# Autodesk Inventor assembly: micromouse
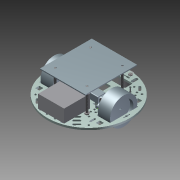
[picture p0: Inventor's stored thumbnail of the model, 180x180]
Saved by Autodesk Inventor 2015 (Build 190159000, 159)
## iProperties
Created: 2015-11-28
Part Number: micromouse
Document SubType Name: Assembly
Designer: user
Author: user
## Documents named in this file (17)
- C:\Users\user\Desktop\UNIVERSIDAD\8 SEMESTRE\FINITOS\Proyecto final\micromouse.iam
- C:\Users\user\Desktop\UNIVERSIDAD\8 SEMESTRE\FINITOS\Proyecto final\Imported Components\bracket\bracket.ipt
- C:\Users\user\Desktop\UNIVERSIDAD\8 SEMESTRE\FINITOS\Proyecto final\Imported Components\PlacaProyectoParaNX_stp\PlacaProyectoParaNX_stp.ipt
- C:\Users\user\Desktop\UNIVERSIDAD\8 SEMESTRE\FINITOS\Proyecto final\Imported Components\micromotor\micromotor.ipt
- C:\Users\user\Desktop\UNIVERSIDAD\8 SEMESTRE\FINITOS\Proyecto final\Imported Components\eje motor\eje motor.ipt
- C:\Users\user\Desktop\UNIVERSIDAD\8 SEMESTRE\FINITOS\Proyecto final\Imported Components\RuedasCaucho\RuedasCaucho.ipt
- C:\Users\user\Desktop\UNIVERSIDAD\8 SEMESTRE\FINITOS\Proyecto final\Imported Components\RuedasCentro\RuedasCentro.ipt
- C:\Users\user\Documents\Inventor\Content Center Files\R2015\es-ES\AS 1112 (4)\AS 1112 - M3(2).ipt
- C:\Users\user\Documents\Inventor\Content Center Files\R2015\es-ES\AS 1427(08)\AS 1427 - M3 x 40(6) I.ipt
- C:\Users\user\Documents\Inventor\Content Center Files\R2015\es-ES\AS 1112 (4)\AS 1112 - M1.6(2).ipt
- C:\Users\user\Documents\Inventor\Content Center Files\R2015\es-ES\BS EN ISO 7045 H\EN ISO 7045 - M1.6 x 12 - 4.8 - H(1).ipt
- C:\Users\user\Desktop\UNIVERSIDAD\8 SEMESTRE\FINITOS\Proyecto final\Imported Components\placa circuito\placa circuito.ipt
- C:\Users\user\Desktop\UNIVERSIDAD\8 SEMESTRE\FINITOS\Proyecto final\bateria.ipt
- C:\Users\user\Desktop\UNIVERSIDAD\8 SEMESTRE\FINITOS\Proyecto final\rueda loca bola.ipt
- C:\Users\user\Desktop\UNIVERSIDAD\8 SEMESTRE\FINITOS\Proyecto final\rueda loca.ipt
- C:\Users\user\Documents\Inventor\Content Center Files\R2015\es-ES\AS 1427(08)\AS 1427 - M2.5 x 25(6) I.ipt
- C:\Users\user\Documents\Inventor\Content Center Files\R2015\es-ES\AS 1112 (4)\AS 1112 - M2.5(2).ipt
## Components (39 placed, 16 different names)
1. bracket:2 — De rotación:1, Rígido:12, Insertar:11, Insertar:12
2. bracket:3 — De rotación:2, Rígido:10, Insertar:13, Insertar:14
3. PlacaProyectoParaNX_stp:1 — De rotación:1, De rotación:2, Insertar:3, Insertar:4, Insertar:5, Insertar:6, Insertar:7, Insertar:9, Insertar:10, Rígido:13, Rígido:14
4. micromotor:1 — Rígido:9, Rígido:12
5. micromotor:2 — Rígido:10, Rígido:11
6. eje motor:1 — Rígido:11, Insertar:1
7. eje motor:2 — Rígido:9, Insertar:2
8. RuedasCaucho:2 — Rígido:7
9. RuedasCentro:3 — Rígido:7, Insertar:1
10. RuedasCaucho:3 — Rígido:8
11. RuedasCentro:4 — Rígido:8, Insertar:2
12. AS 1112 (4) - Métrico M3:1 — Insertar:3
13. AS 1112 (4) - Métrico M3:2 — Insertar:4, Coincidencia:1
14. AS 1112 (4) - Métrico M3:3 — Insertar:5
15. AS 1112 (4) - Métrico M3:4 — Insertar:6
16. AS 1427 Z - Métrico M3 x 40:1 — Insertar:7, Coincidencia:4
17. AS 1427 Z - Métrico M3 x 40:3 — Insertar:9, Coincidencia:3
18. AS 1427 Z - Métrico M3 x 40:4 — Insertar:10, Insertar:20, Coincidencia:2
19. AS 1112 (4) - Métrico M1.6:1 — Insertar:11, Insertar:17
20. AS 1112 (4) - Métrico M1.6:2 — Insertar:12, Insertar:18
21. AS 1112 (4) - Métrico M1.6:3 — Insertar:13, Insertar:16
22. AS 1112 (4) - Métrico M1.6:4 — Insertar:14, Insertar:19
23. BS EN ISO 7045 H - Métrico M1.6 x 12 - 4.8 - H:1 — Insertar:16
24. BS EN ISO 7045 H - Métrico M1.6 x 12 - 4.8 - H:2 — Insertar:17
25. BS EN ISO 7045 H - Métrico M1.6 x 12 - 4.8 - H:3 — Insertar:18
26. BS EN ISO 7045 H - Métrico M1.6 x 12 - 4.8 - H:4 — Insertar:19
27. AS 1427 Z - Métrico M3 x 40:5 — Coincidencia:1, Coincidencia:5
28. placa circuito:1 — Insertar:20
29. AS 1112 (4) - Métrico M3:5 — Coincidencia:2
30. AS 1112 (4) - Métrico M3:6 — Coincidencia:3
31. AS 1112 (4) - Métrico M3:7 — Coincidencia:4
32. AS 1112 (4) - Métrico M3:8 — Coincidencia:5
33. bateria:1 — Rígido:13
34. rueda loca bola:1 — Rígido:15
35. rueda loca:1 — Rígido:14, Rígido:15, Coincidencia:6, Insertar:21
36. AS 1427 Z - Métrico M2.5 x 25:1 — Coincidencia:6, Coincidencia:7
37. AS 1427 Z - Métrico M2.5 x 25:2 — Insertar:21, Coincidencia:8
38. AS 1112 (4) - Métrico M2.5:1 — Coincidencia:7
39. AS 1112 (4) - Métrico M2.5:2 — Coincidencia:8
## Relationships (38: Insert 19, WeldJoint 9, Mate 8, RevoluteJoint 2)
- De rotación:1 [RevoluteJoint]: bracket:2 ↔ PlacaProyectoParaNX_stp:1
- De rotación:2 [RevoluteJoint]: bracket:3 ↔ PlacaProyectoParaNX_stp:1
- Rígido:7 [WeldJoint] (5 mm): RuedasCaucho:2 ↔ RuedasCentro:3
- Rígido:8 [WeldJoint] (5 mm): RuedasCaucho:3 ↔ RuedasCentro:4
- Rígido:9 [WeldJoint]: micromotor:1 ↔ eje motor:2
- Rígido:10 [WeldJoint]: bracket:3 ↔ micromotor:2
- Rígido:11 [WeldJoint]: micromotor:2 ↔ eje motor:1
- Rígido:12 [WeldJoint]: bracket:2 ↔ micromotor:1
- Insertar:1 (-4 mm): eje motor:1 ↔ RuedasCentro:3
- Insertar:2 (-2 mm): eje motor:2 ↔ RuedasCentro:4
- Insertar:3: PlacaProyectoParaNX_stp:1 ↔ AS 1112 (4) - Métrico M3:1
- Insertar:4: PlacaProyectoParaNX_stp:1 ↔ AS 1112 (4) - Métrico M3:2
- Insertar:5: PlacaProyectoParaNX_stp:1 ↔ AS 1112 (4) - Métrico M3:3
- Insertar:6: PlacaProyectoParaNX_stp:1 ↔ AS 1112 (4) - Métrico M3:4
- Insertar:7: PlacaProyectoParaNX_stp:1 ↔ AS 1427 Z - Métrico M3 x 40:1
- Insertar:9: PlacaProyectoParaNX_stp:1 ↔ AS 1427 Z - Métrico M3 x 40:3
- Insertar:10: PlacaProyectoParaNX_stp:1 ↔ AS 1427 Z - Métrico M3 x 40:4
- Insertar:11: bracket:2 ↔ AS 1112 (4) - Métrico M1.6:1
- Insertar:12: bracket:2 ↔ AS 1112 (4) - Métrico M1.6:2
- Insertar:13: bracket:3 ↔ AS 1112 (4) - Métrico M1.6:3
- Insertar:14: bracket:3 ↔ AS 1112 (4) - Métrico M1.6:4
- Insertar:16: AS 1112 (4) - Métrico M1.6:3 ↔ BS EN ISO 7045 H - Métrico M1.6 x 12 - 4.8 - H:1
- Insertar:17: AS 1112 (4) - Métrico M1.6:1 ↔ BS EN ISO 7045 H - Métrico M1.6 x 12 - 4.8 - H:2
- Insertar:18: AS 1112 (4) - Métrico M1.6:2 ↔ BS EN ISO 7045 H - Métrico M1.6 x 12 - 4.8 - H:3
- Insertar:19: AS 1112 (4) - Métrico M1.6:4 ↔ BS EN ISO 7045 H - Métrico M1.6 x 12 - 4.8 - H:4
- Coincidencia:1 [Mate]: AS 1112 (4) - Métrico M3:2 ↔ AS 1427 Z - Métrico M3 x 40:5
- Insertar:20: AS 1427 Z - Métrico M3 x 40:4 ↔ placa circuito:1
- Coincidencia:2 [Mate]: AS 1427 Z - Métrico M3 x 40:4 ↔ AS 1112 (4) - Métrico M3:5
- Coincidencia:3 [Mate]: AS 1427 Z - Métrico M3 x 40:3 ↔ AS 1112 (4) - Métrico M3:6
- Coincidencia:4 [Mate]: AS 1427 Z - Métrico M3 x 40:1 ↔ AS 1112 (4) - Métrico M3:7
- Coincidencia:5 [Mate]: AS 1427 Z - Métrico M3 x 40:5 ↔ AS 1112 (4) - Métrico M3:8
- Rígido:13 [WeldJoint]: PlacaProyectoParaNX_stp:1 ↔ bateria:1
- Rígido:14 [WeldJoint]: PlacaProyectoParaNX_stp:1 ↔ rueda loca:1
- Rígido:15 [WeldJoint]: rueda loca bola:1 ↔ rueda loca:1
- Coincidencia:6 [Mate]: rueda loca:1 ↔ AS 1427 Z - Métrico M2.5 x 25:1
- Insertar:21: rueda loca:1 ↔ AS 1427 Z - Métrico M2.5 x 25:2
- Coincidencia:7 [Mate]: AS 1427 Z - Métrico M2.5 x 25:1 ↔ AS 1112 (4) - Métrico M2.5:1
- Coincidencia:8 [Mate]: AS 1427 Z - Métrico M2.5 x 25:2 ↔ AS 1112 (4) - Métrico M2.5:2
